# Autodesk Inventor assembly: BoltASM
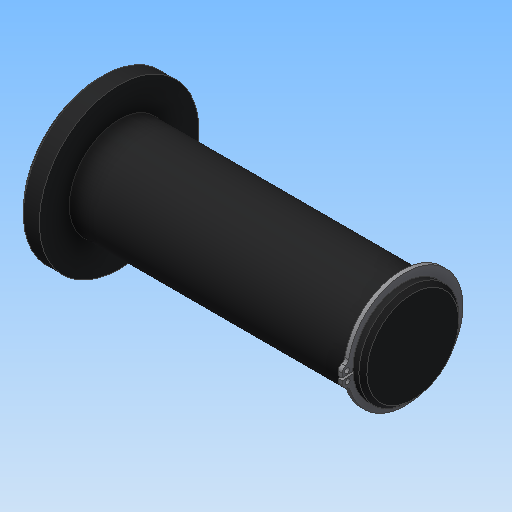
[picture p0: Inventor's stored thumbnail of the model, 512x512]
Saved by Autodesk Inventor 2020.1 (Build 241239000, 239)
## iProperties
Created: 2003-03-06
Part Number: BoltASM
Document SubType Name: Assembly
Designer: rueghs
Control State: 0
Master: False
Checked Out: False
Shininess: 64.0
Length Units: 11269
Angle Units: 11279
Time Units: 11290
Mass Units: 11283
Length Display Precision: 3
Angle Display Precision: 2
Compacted: True
Density: 0.0
Volumn: 0.0
Area: 0.0
PropertySet Name: Model Information
Author: rueghs
## Documents named in this file (3)
- C:\Users\thomastremblay\Desktop\Inventor ACP Data\Assemblies\BoltASM.iam
- C:\Users\thomastremblay\Desktop\Inventor ACP Data\Parts\R-Ring50.ipt
- C:\Users\thomastremblay\Desktop\Inventor ACP Data\Parts\Boltx50.ipt
## Components (2 placed, 2 different names)
1. DIN 471  > 9mm <= 300mm 50 x 2:1 — Insert:1
2. Boltx50:1 — Insert:1
## Relationships (1: Insert 1)
- Insert:1: DIN 471  > 9mm <= 300mm 50 x 2:1 ↔ Boltx50:1
